# Autodesk Inventor assembly: BasicAssembly
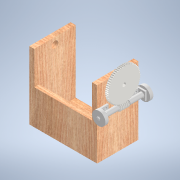
[picture p0: Inventor's stored thumbnail of the model, 180x180]
Saved by Autodesk Inventor 2022.2 (Build 262287010, 287A)
## iProperties
Created: 2022-09-12
Part Number: BasicAssembly
Document SubType Name: Assembly
Designer: robst
Author: robst
## Documents named in this file (6)
- C:\git\CAD-Development\robSteele\ShapeWays\TelescopeProjects\TelescopeMountNov2020\BasicAssembly.iam
- C:\git\CAD-Development\robSteele\ShapeWays\TelescopeProjects\TelescopeMount\woodForkAssembly02.ipt
- C:\git\CAD-Development\robSteele\ShapeWays\TelescopeProjects\TelescopeMount\forkMountForDecTripV01\Design Accelerator\Worm Gears3.iam
- C:\git\CAD-Development\robSteele\ShapeWays\TelescopeProjects\TelescopeMountNov2020\sideSupport.ipt
- C:\git\CAD-Development\robSteele\ShapeWays\TelescopeProjects\TelescopeMountNov2020\3_8 x 7_750-inchHexShaft.ipt
- C:\git\CAD-Development\robSteele\ShapeWays\TelescopeProjects\TelescopeMountNov2020\knobForSideGear.ipt
## Components (7 placed, 5 different names)
1. woodForkAssembly02:1 — Insert:1, Flush:1, Flush:2
2. Worm Gears:1 [sub-assembly] — Insert:1, Insert:2
3. 3_8 x 7_750-inchHexShaft:1 — Insert:2
4. sideSupport:1 — Flush:1, Insert:3
5. sideSupport:2 — Flush:2, Insert:4
6. knobForSideGear:1 — Insert:3
7. knobForSideGear:2 — Insert:4
## Relationships (6: Insert 4, Flush 2)
- Insert:1: woodForkAssembly02:1 ↔ Worm Gears:1
- Insert:2 (-120.65 mm): Worm Gears:1 ↔ 3_8 x 7_750-inchHexShaft:1
- Flush:1: woodForkAssembly02:1 ↔ sideSupport:1
- Flush:2: woodForkAssembly02:1 ↔ sideSupport:2
- Insert:3: sideSupport:1 ↔ knobForSideGear:1
- Insert:4: sideSupport:2 ↔ knobForSideGear:2
